# Autodesk Inventor assembly: MainAssembly
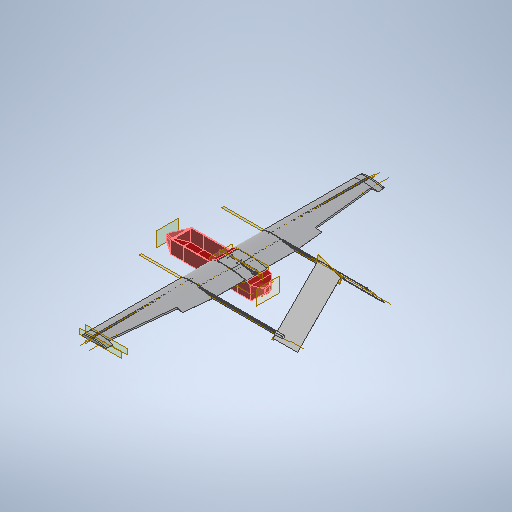
[picture p0: Inventor's stored thumbnail of the model, 512x512]
Saved by Autodesk Inventor 2026 (Build 300175050, 175E)
## iProperties
Created: 2025-07-15
Part Number: MainAssembly
Document SubType Name: Assembly
Designer: Cupri
Author: Cupri
## Documents named in this file (10)
- C:\Users\Cupri\OneDrive - University of South Carolina\Lab projects\UAV\SWIFT-UAV\System_development\Pelican\v0.2\MainAssembly\MainAssembly.iam
- C:\Users\Cupri\OneDrive - University of South Carolina\Lab projects\UAV\SWIFT-UAV\System_development\Pelican\v0.2\SubAssemblies\WingAssembly\WingAssembly.iam
- C:\Users\Cupri\OneDrive - University of South Carolina\Lab projects\UAV\SWIFT-UAV\System_development\Pelican\v0.2\Parts\FuselageParts\EngineSection.ipt
- C:\Users\Cupri\OneDrive - University of South Carolina\Lab projects\UAV\SWIFT-UAV\System_development\Pelican\v0.2\Parts\FuselageParts\WingBoxCouple.ipt
- C:\Users\Cupri\OneDrive - University of South Carolina\Lab projects\UAV\SWIFT-UAV\System_development\Pelican\v0.2\Parts\FuselageParts\ForwardSection.ipt
- C:\Users\Cupri\OneDrive - University of South Carolina\Lab projects\UAV\SWIFT-UAV\System_development\Pelican\v0.2\Parts\FuselageParts\FrontSection.ipt
- C:\Users\Cupri\OneDrive - University of South Carolina\Lab projects\UAV\SWIFT-UAV\System_development\Pelican\v0.2\Parts\Extrusion\20x20x700ExtrudedAluminum.ipt
- C:\Users\Cupri\OneDrive - University of South Carolina\Lab projects\UAV\SWIFT-UAV\System_development\Pelican\v0.2\Parts\Extrusion\20x20x700ExtrudedAluminum_MIR1.ipt
- C:\Users\Cupri\OneDrive - University of South Carolina\Lab projects\UAV\SWIFT-UAV\System_development\Pelican\v0.2\Parts\TailRight.ipt
- C:\Users\Cupri\OneDrive - University of South Carolina\Lab projects\UAV\SWIFT-UAV\System_development\Pelican\v0.2\Parts\TailRight_MIR.ipt
## Components (9 placed, 9 different names)
1. WingAssembly:1 [sub-assembly] — Mate:1, Mate:2, Flush:1, Mate:7, Mate:8, Mate:10
2. 20x20x700ExtrudedAluminum:1 — Mate:7, Mate:8, Mate:10
3. 20x20x700ExtrudedAluminum_MIR1:1 — Mate:11, Mate:12, Mate:13
4. TailRight:1 — Mate:11, Mate:12, Mate:13
5. TailRight_MIR:1
6. EngineSection:1 — Mate:3, Flush:1, Flush:2, Mate:4
7. WingBoxCouple:1 — Mate:1, Mate:2, Mate:3, Flush:2, Mate:4, Mate:5, Flush:4, Mate:9
8. ForwardSection:1 — Mate:5, Flush:4, Mate:6, Flush:8, Flush:9, Mate:9
9. FrontSection:1 — Mate:6, Flush:8, Flush:9
## Relationships (18: Mate 13, Flush 5)
- Mate:1: WingAssembly:1 ↔ WingBoxCouple:1
- Mate:2: WingAssembly:1 ↔ WingBoxCouple:1
- Mate:3: EngineSection:1 ↔ WingBoxCouple:1
- Flush:1: WingAssembly:1 ↔ EngineSection:1
- Flush:2: EngineSection:1 ↔ WingBoxCouple:1
- Mate:4: EngineSection:1 ↔ WingBoxCouple:1
- Mate:5: WingBoxCouple:1 ↔ ForwardSection:1
- Flush:4: WingBoxCouple:1 ↔ ForwardSection:1
- Mate:6: ForwardSection:1 ↔ FrontSection:1
- Flush:8: ForwardSection:1 ↔ FrontSection:1
- Flush:9: ForwardSection:1 ↔ FrontSection:1
- Mate:7: WingAssembly:1 ↔ 20x20x700ExtrudedAluminum:1
- Mate:8: WingAssembly:1 ↔ 20x20x700ExtrudedAluminum:1
- Mate:9: WingBoxCouple:1 ↔ ForwardSection:1
- Mate:10: WingAssembly:1 ↔ 20x20x700ExtrudedAluminum:1
- Mate:11: 20x20x700ExtrudedAluminum_MIR1:1 ↔ TailRight:1
- Mate:12: 20x20x700ExtrudedAluminum_MIR1:1 ↔ TailRight:1
- Mate:13: 20x20x700ExtrudedAluminum_MIR1:1 ↔ TailRight:1
